# Autodesk Inventor assembly: bearing_flat_w_hardware_offset
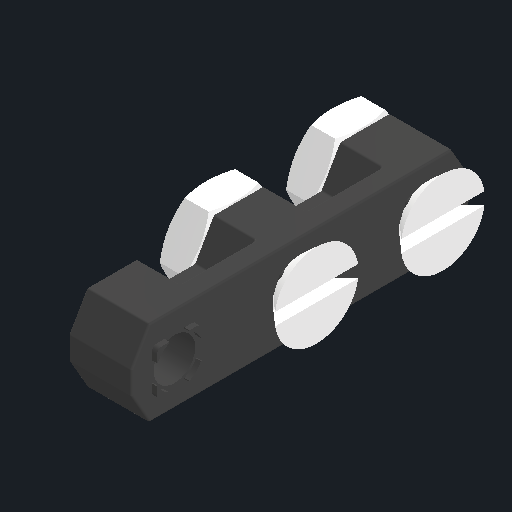
[picture p0: Inventor's stored thumbnail of the model, 512x512]
Saved by Autodesk Inventor 2025 (Build 290162000, 162)
## iProperties
Created: 2024-10-10
Part Number: bearing_flat_w_hardware_offset
Document SubType Name: Assembly
Designer: Averey Ku
Author: Averey Ku
## Documents named in this file (5)
- D:\vex_robotics_high_stakes\hardware\cad\robpros_cad_lib\Quick Assemblies\bearing_flat_w_hardware_offset.iam
- D:\vex_robotics_high_stakes\hardware\cad\robpros_cad_lib\Structure\Hardware\Screw Nylon - Slotted\NScrew Slotted Threaded .500.ipt
- D:\vex_robotics_high_stakes\hardware\cad\robpros_cad_lib\Motion\Shaft LS\Bearing Flat Low Profile.ipt
- D:\vex_robotics_high_stakes\hardware\cad\robpros_cad_lib\Structure\Hardware\Nut Nylon\Nut Nylon - White.ipt
- D:\vex_robotics_high_stakes\hardware\cad\robpros_cad_lib\Structure\Hardware\Nut Nylon.ipt
## Components (5 placed, 3 different names)
1. NScrew Slotted Threaded .500:1 — Insert:5
2. NScrew Slotted Threaded .500:2 — Insert:2
3. Bearing Flat Low Profile:1 — Insert:2, Insert:4, Insert:5, Insert:6
4. Nut Nylon - White:1 — Insert:4
5. Nut Nylon - White:2 — Insert:6
## Relationships (4: Insert 4)
- Insert:2 (-1.5875 mm): NScrew Slotted Threaded .500:2 ↔ Bearing Flat Low Profile:1
- Insert:4 (1.27 mm): Bearing Flat Low Profile:1 ↔ Nut Nylon - White:1
- Insert:5 (-1.5875 mm): NScrew Slotted Threaded .500:1 ↔ Bearing Flat Low Profile:1
- Insert:6 (1.27 mm): Bearing Flat Low Profile:1 ↔ Nut Nylon - White:2
